# Autodesk Inventor assembly: case_construct
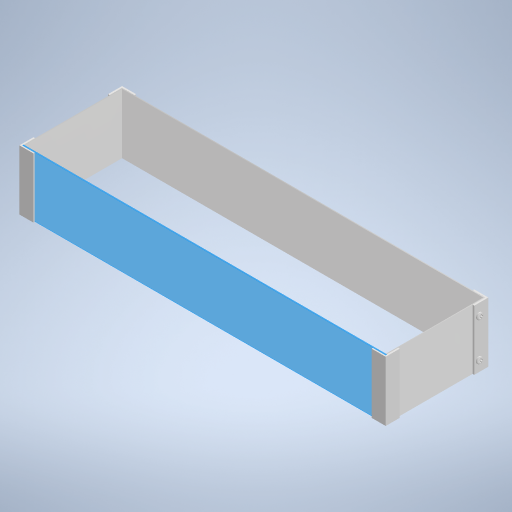
[picture p0: Inventor's stored thumbnail of the model, 512x512]
Saved by Autodesk Inventor 2023 (Build 270158000, 158)
## iProperties
Created: 2022-09-22
Part Number: case_construct
Document SubType Name: Assembly
Designer: Desmond
Author: Desmond
## Documents named in this file (5)
- G:\LED Nixie Test\Glass Tube\case_construct.iam
- G:\LED Nixie Test\Glass Tube\side_case_v2.ipt
- G:\LED Nixie Test\Glass Tube\side_case_v2_2.ipt
- G:\LED Nixie Test\Glass Tube\corners.ipt
- G:\m3x6-philips-head-screw-1.snapshot.5\M3x6 Philips Screw.ipt
## Components (12 placed, 4 different names)
1. side_case_v2:1 — Mate:2, Mate:3, Flush:2, Flush:3, Flush:4, Mate:7, Flush:10, Flush:13, Mate:10
2. side_case_v2:2 — Mate:1, Mate:4, Flush:1, Flush:5, Flush:6, Flush:7, Flush:8, Mate:5, Flush:11, Flush:12, Mate:8
3. side_case_v2_2:1 — Mate:3, Mate:4, Flush:3, Flush:4, Flush:5, Mate:9, Mate:11
4. side_case_v2_2:2 — Mate:1, Mate:2, Flush:1, Flush:2, Flush:6, Mate:6, Mate:16
5. corners:1 — Flush:7, Flush:8, Mate:5, Mate:6
6. corners:2 — Flush:13, Mate:10, Mate:11
7. corners:3 — Mate:7, Flush:10, Mate:12, Mate:13, Mate:14, Mate:15, Mate:16
8. corners:4 — Flush:11, Flush:12, Mate:8, Mate:9
9. M3x6 Philips Screw:5 — Mate:13
10. M3x6 Philips Screw:6 — Mate:12
11. M3x6 Philips Screw:7 — Mate:14
12. M3x6 Philips Screw:8 — Mate:15
## Relationships (28: Mate 16, Flush 12)
- Mate:1: side_case_v2:2 ↔ side_case_v2_2:2
- Mate:2: side_case_v2:1 ↔ side_case_v2_2:2
- Mate:3: side_case_v2:1 ↔ side_case_v2_2:1
- Mate:4: side_case_v2:2 ↔ side_case_v2_2:1
- Flush:1: side_case_v2:2 ↔ side_case_v2_2:2
- Flush:2: side_case_v2:1 ↔ side_case_v2_2:2
- Flush:3: side_case_v2:1 ↔ side_case_v2_2:1
- Flush:4: side_case_v2:1 ↔ side_case_v2_2:1
- Flush:5: side_case_v2:2 ↔ side_case_v2_2:1
- Flush:6: side_case_v2:2 ↔ side_case_v2_2:2
- Flush:7: side_case_v2:2 ↔ corners:1
- Flush:8: side_case_v2:2 ↔ corners:1
- Mate:5: side_case_v2:2 ↔ corners:1
- Mate:6: side_case_v2_2:2 ↔ corners:1
- Mate:7: side_case_v2:1 ↔ corners:3
- Flush:10: side_case_v2:1 ↔ corners:3
- Flush:11: side_case_v2:2 ↔ corners:4
- Flush:12: side_case_v2:2 ↔ corners:4
- Mate:8: side_case_v2:2 ↔ corners:4
- Mate:9: side_case_v2_2:1 ↔ corners:4
- Flush:13: side_case_v2:1 ↔ corners:2
- Mate:10: side_case_v2:1 ↔ corners:2
- Mate:11: side_case_v2_2:1 ↔ corners:2
- Mate:12: corners:3 ↔ M3x6 Philips Screw:6
- Mate:13: corners:3 ↔ M3x6 Philips Screw:5
- Mate:14: corners:3 ↔ M3x6 Philips Screw:7
- Mate:15: corners:3 ↔ M3x6 Philips Screw:8
- Mate:16: side_case_v2_2:2 ↔ corners:3
